# Autodesk Inventor assembly: ASY MSC 900.5 BASE FRAME
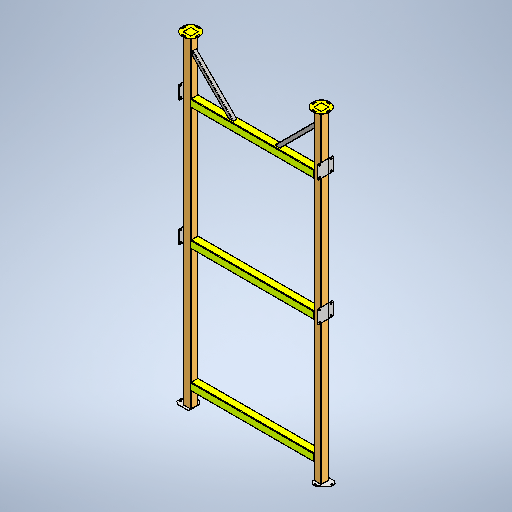
[picture p0: Inventor's stored thumbnail of the model, 512x512]
Saved by Autodesk Inventor 2025 (Build 290162010, 162A)
## iProperties
_SolveAssemblyDoc: Frame Generator Solve Assembly
_Version: 25.0.0
Created: 2024-06-27
Part Number: ASY MSC 900.5 BASE FRAME
Document SubType Name: Assembly
Designer: admin
Stock Number: МОО 900.5 базовая рама 2
Author: admin
## Documents named in this file (7)
- C:\Users\admin\YandexDisk-badmisterfox\домашниий пк\Inventor\Manturovo\Manturovo_Se-clar\Pillars\ASY MSC 900.5 base frame.iam
- C:\Users\admin\YandexDisk-badmisterfox\домашниий пк\Inventor\Manturovo\Manturovo_Se-clar\MSC DIM 009.5 base frame sketch.ipt
- C:\Users\admin\YandexDisk-badmisterfox\домашниий пк\Inventor\Manturovo\Manturovo_Se-clar\Pillars\ASY MSC 900.5.1 base frame.iam
- C:\Users\admin\YandexDisk-badmisterfox\домашниий пк\Inventor\Manturovo\Manturovo_Se-clar\MSC DIM 001 frame.ipt
- C:\Users\admin\YandexDisk-badmisterfox\домашниий пк\Inventor\Manturovo\Manturovo_Se-clar\MSC 902 flange frame heel.ipt
- C:\Users\admin\YandexDisk-badmisterfox\домашниий пк\Inventor\Manturovo\Manturovo_Se-clar\MSC 906 flange frame.ipt
- C:\Users\admin\YandexDisk-badmisterfox\домашниий пк\Inventor\Manturovo\Manturovo_Se-clar\MSC 908 transverse pillar plate.ipt
## Components (10 placed, 5 different names)
1. MSC DIM 009.5 base frame sketch.ipt:1 — Mate:1, Flush:1, Flush:2
2. ASY MSC 900.5.1 base frame.iam:1 [sub-assembly] — Rigid:3, Rigid:4, Rigid:5, Rigid:6, Mate:2, Flush:3, Mate:4, Mate:6
3. MSC 902 flange frame heel.ipt:1 — Rigid:5
4. MSC 902 flange frame heel.ipt:2 — Rigid:6, Mate:3, Mate:5
5. MSC 906 flange frame.ipt:1 — Rigid:3
6. MSC 906 flange frame.ipt:2 — Rigid:4
7. MSC 908 transverse pillar plate.ipt:1 — Rigid:11
8. MSC 908 transverse pillar plate.ipt:2 — Rigid:12
9. MSC 908 transverse pillar plate.ipt:3 — Mate:2, Mate:3, Flush:3, Rigid:11
10. MSC 908 transverse pillar plate.ipt:4 — Mate:4, Mate:5, Mate:6, Rigid:12
## Relationships (15: WeldJoint 6, Mate 6, Flush 3)
- Rigid:3 [WeldJoint]: ASY MSC 900.5.1 base frame.iam:1 ↔ MSC 906 flange frame.ipt:1
- Rigid:4 [WeldJoint]: ASY MSC 900.5.1 base frame.iam:1 ↔ MSC 906 flange frame.ipt:2
- Rigid:5 [WeldJoint]: ASY MSC 900.5.1 base frame.iam:1 ↔ MSC 902 flange frame heel.ipt:1
- Rigid:6 [WeldJoint]: ASY MSC 900.5.1 base frame.iam:1 ↔ MSC 902 flange frame heel.ipt:2
- Mate:1: MSC DIM 009.5 base frame sketch.ipt:1
- Flush:1: MSC DIM 009.5 base frame sketch.ipt:1
- Flush:2: MSC DIM 009.5 base frame sketch.ipt:1
- Mate:2: ASY MSC 900.5.1 base frame.iam:1 ↔ MSC 908 transverse pillar plate.ipt:3
- Mate:3 (2736 mm): MSC 902 flange frame heel.ipt:2 ↔ MSC 908 transverse pillar plate.ipt:3
- Flush:3: ASY MSC 900.5.1 base frame.iam:1 ↔ MSC 908 transverse pillar plate.ipt:3
- Rigid:11 [WeldJoint] (1425 mm): MSC 908 transverse pillar plate.ipt:1 ↔ MSC 908 transverse pillar plate.ipt:3
- Mate:4: ASY MSC 900.5.1 base frame.iam:1 ↔ MSC 908 transverse pillar plate.ipt:4
- Mate:5 (1446 mm): MSC 902 flange frame heel.ipt:2 ↔ MSC 908 transverse pillar plate.ipt:4
- Mate:6: ASY MSC 900.5.1 base frame.iam:1 ↔ MSC 908 transverse pillar plate.ipt:4
- Rigid:12 [WeldJoint] (1425 mm): MSC 908 transverse pillar plate.ipt:2 ↔ MSC 908 transverse pillar plate.ipt:4
## Named parameters: frame_1 = 334.24956 mm, frame_3 = 2905.4 mm, frame_4 = 4190.97522 mm, frame_5 = 5476.55043 mm, Ширина_рамы = 1425 mm, Отступ_до_ниж_перекладины = 160 mm, Отступ_до_сред_перекладины = 1510 mm, Шаг_опор_по_баку = 2000 mm, Движение_рамы_вперед_назад = 270 mm, frame_2 = 1619.82478 mm, frame_6 = 6762.12565 mm, Высота_опорных_стоек = 151 mm
